# Autodesk Inventor assembly: Assem
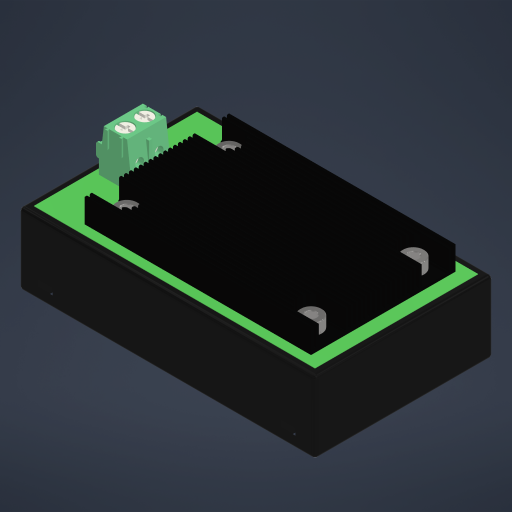
[picture p0: Inventor's stored thumbnail of the model, 512x512]
Saved by Autodesk Inventor 2023.2 (Build 272271000, 271)
## iProperties
Created: 2023-01-15
Part Number: Assem
Document SubType Name: Assembly
Designer: adnew
Sending System: SolidWorks 2022
Last Author: AdamNewhouse
Last Saved: 2023-01-15
Definition: design
Part Number: coprocessor-psu 1
Nomenclature: coprocessor-psu 1
Author: adnew
## Documents named in this file (5)
- C:\Users\adnew\git\coprocessor-psu\3d\Assem\Assem.iam
- C:\Users\adnew\git\coprocessor-psu\3d\Assem\HEATSINK.ipt
- C:\Users\adnew\git\coprocessor-psu\3d\Assem\90751A110_18-8 Stainless Steel Socket Head Screws.ipt
- C:\Users\adnew\git\coprocessor-psu\3d\coprocessor-psu\coprocessor-psu.iam
- C:\Users\adnew\git\coprocessor-psu\3d\case.ipt
## Components (7 placed, 4 different names)
1. HEATSINK:1 — Insert:1, Insert:2
2. 90751A110_18-8 Stainless Steel Socket Head Screws:1
3. 90751A110_18-8 Stainless Steel Socket Head Screws:2
4. 90751A110_18-8 Stainless Steel Socket Head Screws:3
5. 90751A110_18-8 Stainless Steel Socket Head Screws:4
6. coprocessor-psu:1 [sub-assembly] — Insert:1, Insert:2, Flush:1
7. case:1 — Flush:1
## Relationships (3: Insert 2, Flush 1)
- Insert:1: HEATSINK:1 ↔ coprocessor-psu:1
- Insert:2: HEATSINK:1 ↔ coprocessor-psu:1
- Flush:1: coprocessor-psu:1 ↔ case:1
